# Autodesk Inventor assembly: Общая сборка
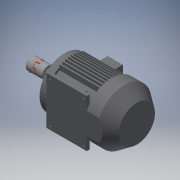
[picture p0: Inventor's stored thumbnail of the model, 180x180]
Saved by Autodesk Inventor 2016 (Build 200138000, 138)
## iProperties
Created: 2021-04-30
Part Number: Общая сборка
Material: Типовые
Document SubType Name: Assembly
Designer: Лол
Author: Лол
## Documents named in this file (3)
- C:\Users\Лол\Documents\Inventor\course_work\Общая сборка.iam
- C:\Users\Лол\Documents\Inventor\course_work\Электродвигатель АИР132M2,4,6,8.ipt
- C:\Users\Лол\Documents\Inventor\course_work\Муфта двигателя.iam
## Components (2 placed, 2 different names)
1. Электродвигатель АИР132M2,4,6,8:1 — Совмещение:1, Совмещение:2, Совмещение:3, Допуск симметричности:1
2. Муфта двигателя:1 [sub-assembly] — Совмещение:1, Совмещение:2, Совмещение:3, Допуск симметричности:1
## Relationships (4: Mate 3, Symmetry 1)
- Совмещение:1 [Mate]: Электродвигатель АИР132M2,4,6,8:1 ↔ Муфта двигателя:1
- Совмещение:2 [Mate]: Электродвигатель АИР132M2,4,6,8:1 ↔ Муфта двигателя:1
- Совмещение:3 [Mate] (-30 mm): Электродвигатель АИР132M2,4,6,8:1 ↔ Муфта двигателя:1
- Допуск симметричности:1 [Symmetry]: Электродвигатель АИР132M2,4,6,8:1 ↔ Муфта двигателя:1
